# Autodesk Inventor assembly: ASY mixer1
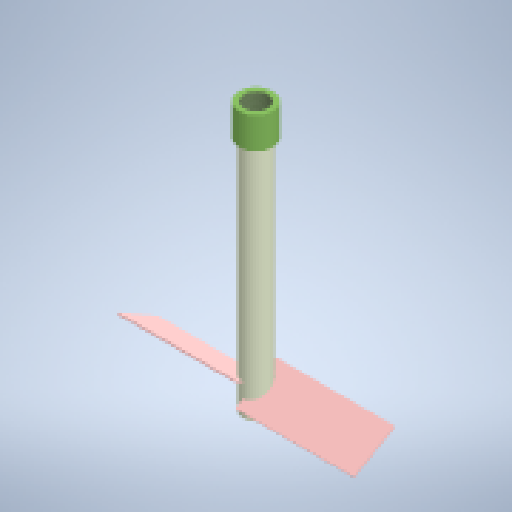
[picture p0: Inventor's stored thumbnail of the model, 512x512]
Saved by Autodesk Inventor 2023.1 (Build 271208000, 208)
## iProperties
Created: 2023-08-07
Part Number: ASY mixer1
Document SubType Name: Assembly
Designer: admin
Author: admin
## Documents named in this file (4)
- C:\Users\admin\My Drive (bigstupidbeast@gmail.com)\Inventor\StoTSy Furmanovo\CAD\Mixer 1\ASY mixer1.iam
- C:\Users\admin\My Drive (bigstupidbeast@gmail.com)\Inventor\StoTSy Furmanovo\CAD\Mixer 1\mixer ring 1.ipt
- C:\Users\admin\My Drive (bigstupidbeast@gmail.com)\Inventor\StoTSy Furmanovo\CAD\Mixer 1\vane mixer.ipt
- C:\Users\admin\My Drive (bigstupidbeast@gmail.com)\Inventor\StoTSy Furmanovo\CAD\Mixer 1\bush mixer.ipt
## Components (4 placed, 3 different names)
1. mixer ring 1:1 — Rigid:1, Rigid:2
2. vane mixer:1 — Flush:1, Rigid:1
3. vane mixer:2 — Rigid:2
4. bush mixer:1
## Relationships (4: WeldJoint 3, Flush 1)
- Flush:1: vane mixer:1
- Rigid:1 [WeldJoint] (-30 mm): mixer ring 1:1 ↔ vane mixer:1
- Rigid:2 [WeldJoint] (-30 mm): mixer ring 1:1 ↔ vane mixer:2
- [WeldJoint]: mixer ring 1:1 ↔ bush mixer:1
